# Autodesk Inventor assembly: Assembly4
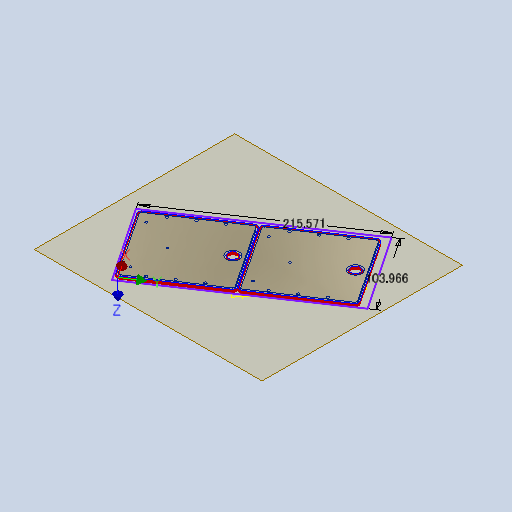
[picture p0: Inventor's stored thumbnail of the model, 512x512]
Saved by Autodesk Inventor 2025.2 (Build 292293000, 293)
## iProperties
Created: 2024-12-16
Part Number: Assembly4
Document SubType Name: Assembly
Designer: haruy
Author: haruy
## Documents named in this file (2)
- C:\Users\haruy\Documents\ロボコン\NHK2025\cad\cnc\Assembly4.iam
- C:\Users\haruy\Documents\ロボコン\NHK2025\cad\nagahisa\belt_liner\belt_liner_v1_Plate_3.ipt
## Components (2 placed, 1 different names)
1. belt_liner_v1_Plate_3:1 — フラッシュ:1, フラッシュ:3, メイト:1
2. belt_liner_v1_Plate_3:2 — フラッシュ:2, フラッシュ:3, メイト:1
## Relationships (4: Flush 3, Mate 1)
- フラッシュ:1 [Flush]: belt_liner_v1_Plate_3:1
- フラッシュ:2 [Flush]: belt_liner_v1_Plate_3:2
- フラッシュ:3 [Flush]: belt_liner_v1_Plate_3:1 ↔ belt_liner_v1_Plate_3:2
- メイト:1 [Mate] (5 mm): belt_liner_v1_Plate_3:1 ↔ belt_liner_v1_Plate_3:2
